# Autodesk Inventor assembly: MAX Axel Hub
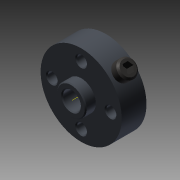
[picture p0: Inventor's stored thumbnail of the model, 180x180]
Saved by Autodesk Inventor 2015 (Build 190159000, 159)
## iProperties
Created: 2015-10-21
Part Number: MAX Axel Hub
Document SubType Name: Assembly
Designer: Mason
Author: Mason
## Documents named in this file (3)
- C:\Users\Mason\Documents\Inventor\Content Center Files\FTC\MAX Axel Hub.iam
- C:\Users\Public\Documents\Autodesk\Vault Basic 2015\Samples\Inventor 2014\Padlock\Designs\Imported Components\tetrix_739172_2012\TETRIX_739172_COLLAR_2012.ipt
- C:\Users\Public\Documents\Autodesk\Vault Basic 2015\Samples\Inventor 2014\Padlock\Designs\Imported Components\tetrix_739172_2012\TETRIX_739172_SCREW_2012.ipt
## Components (2 placed, 2 different names)
1. TETRIX_739172_COLLAR_2012:1 — Mate:1
2. TETRIX_739172_SCREW_2012:1 — Mate:1
## Relationships (1: Mate 1)
- Mate:1: TETRIX_739172_COLLAR_2012:1 ↔ TETRIX_739172_SCREW_2012:1
